# Autodesk Inventor assembly: Wheel on a Stick
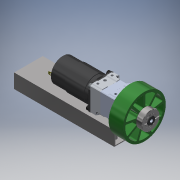
[picture p0: Inventor's stored thumbnail of the model, 180x180]
Saved by Autodesk Inventor 2018 (Build 220112000, 112)
## iProperties
Created: 2020-01-28
Part Number: Wheel on a Stick
Document SubType Name: Assembly
Designer: maste
Author: maste
## Documents named in this file (7)
- \\studenthome\students\S-2512711\GitHub\2020CAD\Control panel spinny boi\Main Assembly File\Wheel on a Stick.iam
- \\studenthome\students\S-2512711\GitHub\2020CAD\Control panel spinny boi\Part Files\VersaPlanetary_v2_Single_Stage_10_1_with_775_Series.iam
- \\studenthome\students\S-2512711\GitHub\2020CAD\Control panel spinny boi\Part Files\am-3945 3IN 500Hex Compliant Wheel VER 3.ipt
- \\studenthome\students\S-2512711\GitHub\2020CAD\Control panel spinny boi\Part Files\am-1526 500Hex HD Collar Clamp.iam
- \\studenthome\students\S-2512711\GitHub\2020CAD\Control panel spinny boi\Part Files\0.0625 Hex Spacer.ipt
- \\studenthome\students\S-2512711\GitHub\2020CAD\Control panel spinny boi\Part Files\1x2 Placeholder.ipt
- \\studenthome\students\S-2512711\GitHub\2020CAD\Control panel spinny boi\Part Files\92196A276_18-8 STAINLESS STEEL SOCKET HEAD CAP SCREW.ipt
## Components (9 placed, 6 different names)
1. VersaPlanetary_v2_Single_Stage_10_1_with_775_Series:1 [sub-assembly] — Mate:1, Mate:2, Mate:3, Mate:4, Flush:1, Mate:6, Mate:7, Mate:8, Mate:9, Mate:10, Mate:11
2. am-3945 3IN 500Hex Compliant Wheel VER 3:1 — Mate:1, Mate:2, Mate:5
3. am-1526 500Hex HD Collar Clamp:1 [sub-assembly] — Mate:3, Mate:4, Flush:1, Mate:5
4. 0.0625 Hex Spacer:1 — Mate:6, Mate:7, Mate:8
5. 1x2 Placeholder:1 — Mate:9, Mate:10, Mate:11, Mate:12, Mate:13, Mate:14, Mate:15, Mate:16, Mate:17, Mate:18, Mate:19, Rotation:1, Rotation:2, Rotation:3, Rotation:4
6. 92196A276_18-8 STAINLESS STEEL SOCKET HEAD CAP SCREW:1 — Mate:14, Mate:19, Rotation:4
7. 92196A276_18-8 STAINLESS STEEL SOCKET HEAD CAP SCREW:2 — Mate:12, Mate:13, Rotation:1
8. 92196A276_18-8 STAINLESS STEEL SOCKET HEAD CAP SCREW:3 — Mate:16, Mate:17, Rotation:2
9. 92196A276_18-8 STAINLESS STEEL SOCKET HEAD CAP SCREW:4 — Mate:15, Mate:18, Rotation:3
## Relationships (24: Mate 19, RelateRotation 4, Flush 1)
- Mate:1: VersaPlanetary_v2_Single_Stage_10_1_with_775_Series:1 ↔ am-3945 3IN 500Hex Compliant Wheel VER 3:1
- Mate:2: VersaPlanetary_v2_Single_Stage_10_1_with_775_Series:1 ↔ am-3945 3IN 500Hex Compliant Wheel VER 3:1
- Mate:3: VersaPlanetary_v2_Single_Stage_10_1_with_775_Series:1 ↔ am-1526 500Hex HD Collar Clamp:1
- Mate:4: VersaPlanetary_v2_Single_Stage_10_1_with_775_Series:1 ↔ am-1526 500Hex HD Collar Clamp:1
- Flush:1: VersaPlanetary_v2_Single_Stage_10_1_with_775_Series:1 ↔ am-1526 500Hex HD Collar Clamp:1
- Mate:5: am-3945 3IN 500Hex Compliant Wheel VER 3:1 ↔ am-1526 500Hex HD Collar Clamp:1
- Mate:6: VersaPlanetary_v2_Single_Stage_10_1_with_775_Series:1 ↔ 0.0625 Hex Spacer:1
- Mate:7: VersaPlanetary_v2_Single_Stage_10_1_with_775_Series:1 ↔ 0.0625 Hex Spacer:1
- Mate:8: VersaPlanetary_v2_Single_Stage_10_1_with_775_Series:1 ↔ 0.0625 Hex Spacer:1
- Mate:9: VersaPlanetary_v2_Single_Stage_10_1_with_775_Series:1 ↔ 1x2 Placeholder:1
- Mate:10: VersaPlanetary_v2_Single_Stage_10_1_with_775_Series:1 ↔ 1x2 Placeholder:1
- Mate:11: VersaPlanetary_v2_Single_Stage_10_1_with_775_Series:1 ↔ 1x2 Placeholder:1
- Mate:12: 1x2 Placeholder:1 ↔ 92196A276_18-8 STAINLESS STEEL SOCKET HEAD CAP SCREW:2
- Mate:13: 1x2 Placeholder:1 ↔ 92196A276_18-8 STAINLESS STEEL SOCKET HEAD CAP SCREW:2
- Mate:14: 1x2 Placeholder:1 ↔ 92196A276_18-8 STAINLESS STEEL SOCKET HEAD CAP SCREW:1
- Mate:15: 1x2 Placeholder:1 ↔ 92196A276_18-8 STAINLESS STEEL SOCKET HEAD CAP SCREW:4
- Mate:16: 1x2 Placeholder:1 ↔ 92196A276_18-8 STAINLESS STEEL SOCKET HEAD CAP SCREW:3
- Mate:17: 1x2 Placeholder:1 ↔ 92196A276_18-8 STAINLESS STEEL SOCKET HEAD CAP SCREW:3
- Mate:18: 1x2 Placeholder:1 ↔ 92196A276_18-8 STAINLESS STEEL SOCKET HEAD CAP SCREW:4
- Mate:19: 1x2 Placeholder:1 ↔ 92196A276_18-8 STAINLESS STEEL SOCKET HEAD CAP SCREW:1
- Rotation:1 [RelateRotation] (1 ul): 1x2 Placeholder:1 ↔ 92196A276_18-8 STAINLESS STEEL SOCKET HEAD CAP SCREW:2
- Rotation:2 [RelateRotation] (1 ul): 1x2 Placeholder:1 ↔ 92196A276_18-8 STAINLESS STEEL SOCKET HEAD CAP SCREW:3
- Rotation:3 [RelateRotation] (1 ul): 1x2 Placeholder:1 ↔ 92196A276_18-8 STAINLESS STEEL SOCKET HEAD CAP SCREW:4
- Rotation:4 [RelateRotation] (1 ul): 1x2 Placeholder:1 ↔ 92196A276_18-8 STAINLESS STEEL SOCKET HEAD CAP SCREW:1
